# Autodesk Inventor assembly: wheel assembly.reinvented2
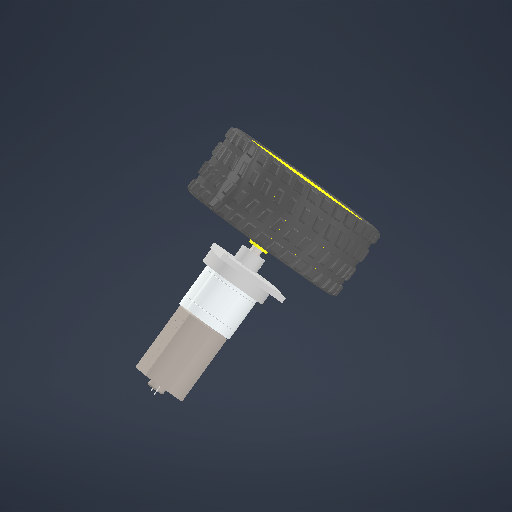
[picture p0: Inventor's stored thumbnail of the model, 512x512]
Saved by Autodesk Inventor 2027 (Build 310192000, 192)
## iProperties
Created: 2026-06-27
Part Number: wheel assembly.reinvented2
Document SubType Name: Assembly
Designer: uchiha
Author: uchiha
## Documents named in this file (5)
- C:\Users\uchiha\Desktop\New folder\designdj\New folder\wheel assembly.reinvented2.iam
- C:\Users\uchiha\Desktop\New folder\designdj\parts\20d-metal-gearmotors-3d-models\20d-metal-gearmotor-63-78\20d-metal-gearmotor-63-78.ipt
- C:\Users\uchiha\Desktop\New folder\designdj\motorassembly.ipt
- C:\Users\uchiha\Desktop\New folder\designdj\rocker-bogie-mechanism-mars-rover-1.snapshot.9\assembly\wheel.ipt
- C:\Users\uchiha\Desktop\New folder\designdj\New folder\motorbracket.ipt
## Components (4 placed, 4 different names)
1. 20d-metal-gearmotor-63-78:1 — Mate:1, Mate:5, Mate:6, Mate:7, Mate:8, Insert:1, Rotation:1, Rotation:2
2. wheel:1 — Mate:8, Insert:1, Rotation:1, Rotation:2
3. motorbracket:1 — Mate:5, Mate:6, Mate:7
4. motorassembly:1 — Mate:1
## Relationships (8: Mate 5, RelateRotation 2, Insert 1)
- Mate:1: 20d-metal-gearmotor-63-78:1 ↔ motorassembly:1
- Mate:5: 20d-metal-gearmotor-63-78:1 ↔ motorbracket:1
- Mate:6: 20d-metal-gearmotor-63-78:1 ↔ motorbracket:1
- Mate:7: 20d-metal-gearmotor-63-78:1 ↔ motorbracket:1
- Mate:8: 20d-metal-gearmotor-63-78:1 ↔ wheel:1
- Insert:1 (-6 mm): 20d-metal-gearmotor-63-78:1 ↔ wheel:1
- Rotation:1 [RelateRotation] (1 ul): 20d-metal-gearmotor-63-78:1 ↔ wheel:1
- Rotation:2 [RelateRotation] (1 ul): 20d-metal-gearmotor-63-78:1 ↔ wheel:1
